# Autodesk Inventor assembly: V1Indexers
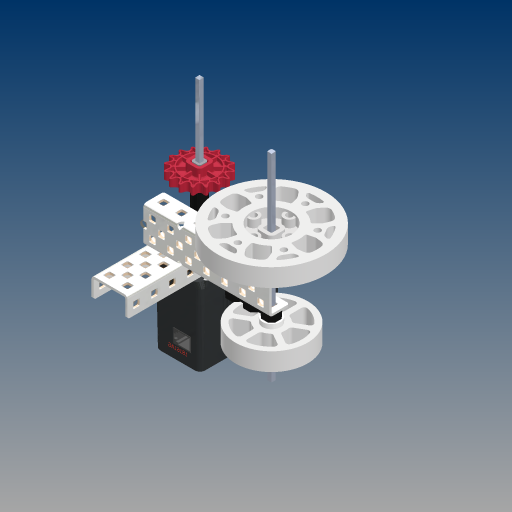
[picture p0: Inventor's stored thumbnail of the model, 512x512]
Saved by Autodesk Inventor 2023 (Build 270158000, 158)
## iProperties
Created: 2023-07-14
Part Number: V1Indexers
Document SubType Name: Assembly
Designer: eddie
Author: eddie
## Documents named in this file (20)
- C:\Users\eddie\Documents\81208X-Over-Under-CAD\V1\V1Indexer_Right.iam
- C:\Users\eddie\Documents\81208X-Over-Under-CAD\VEX-CAD-Inventor-1.4.0\Motion\Shaft LS\Shaft LS.ipt
- C:\Users\eddie\Documents\81208X-Over-Under-CAD\VEX-CAD-Inventor-1.4.0\Motion\Spacers\Spacer Nylon .375 OD\NSpacer .375 OD x .500.ipt
- C:\Users\eddie\Documents\81208X-Over-Under-CAD\VEX-CAD-Inventor-1.4.0\Motion\Spacers\Spacer Nylon .375 OD.ipt
- C:\Users\eddie\Documents\81208X-Over-Under-CAD\VEX-CAD-Inventor-1.4.0\Motion\Shaft LS\Shaft LS\Shaft LS 3.5.ipt
- C:\Users\eddie\Documents\81208X-Over-Under-CAD\VEX-CAD-Inventor-1.4.0\Motion\Shaft LS\Shaft LS\Shaft LS 5.5.ipt
- C:\Users\eddie\Documents\81208X-Over-Under-CAD\VEX-CAD-Inventor-1.4.0\Motion\Spacers\Spacer Nylon .500 OD\NSpacer White .500 OD x .125.ipt
- C:\Users\eddie\Documents\81208X-Over-Under-CAD\VEX-CAD-Inventor-1.4.0\Motion\Spacers\Spacer Nylon .500 OD.ipt
- C:\Users\eddie\Documents\81208X-Over-Under-CAD\VEX-CAD-Inventor-1.4.0\Motion\Wheels\Flex Wheels\2.000 Flex Wheel\2.000 30A .500.ipt
- C:\Users\eddie\Documents\81208X-Over-Under-CAD\VEX-CAD-Inventor-1.4.0\Motion\Wheels\Flex Wheels\2.000 Flex Wheel.ipt
- C:\Users\eddie\Documents\81208X-Over-Under-CAD\VEX-CAD-Inventor-1.4.0\Motion\Wheels\Flex Wheels\3.000 Flex Wheel\3.000 30A .500.ipt
- C:\Users\eddie\Documents\81208X-Over-Under-CAD\VEX-CAD-Inventor-1.4.0\Motion\Wheels\Flex Wheels\3.000 Flex Wheel.ipt
- C:\Users\eddie\Documents\81208X-Over-Under-CAD\VEX-CAD-Inventor-1.4.0\Structure\C Channel\Aluminum 1x2x1\Alu C 1x2x1x9_MIR1.ipt
- C:\Users\eddie\Documents\81208X-Over-Under-CAD\VEX-CAD-Inventor-1.4.0\Motion\Shaft LS\Bearing Flat_MIR2.ipt
- C:\Users\eddie\Documents\81208X-Over-Under-CAD\VEX-CAD-Inventor-1.4.0\Structure\C Channel\Aluminum 1x2x1\Alu C 1x2x1x7_MIR1.ipt
- C:\Users\eddie\Documents\81208X-Over-Under-CAD\VEX-CAD-Inventor-1.4.0\Electronics\V5 Motor_MIR1.ipt
- C:\Users\eddie\Documents\81208X-Over-Under-CAD\VEX-CAD-Inventor-1.4.0\Motion\Sprockets\6P Sprocket\6P 16T Sprocket, Square_MIR1.iam
- C:\Users\eddie\Documents\81208X-Over-Under-CAD\VEX-CAD-Inventor-1.4.0\Motion\Sprockets\6P Sprocket\6P 8T Sprocket, Square_MIR1.iam
- C:\Users\eddie\Documents\81208X-Over-Under-CAD\VEX-CAD-Inventor-1.4.0\Motion\Gears\HS Gear\HS 12T Gear, Square_MIR1.iam
- C:\Users\eddie\Documents\81208X-Over-Under-CAD\Custom-parts\36T HS Gear Insert_MIR_MIR.ipt
## Components (17 placed, 14 different names)
1. Alu C 1x2x1x9_MIR1:1 — Insert:40, Insert:41
2. Bearing Flat_MIR2:1 — Insert:40, Insert:42, Insert:45, Insert:46
3. Alu C 1x2x1x7_MIR1:1 — Insert:41, Insert:43, Insert:44, Insert:49, Insert:51
4. V5 Motor_MIR1:1 — Insert:42
5. Shaft LS 5.5:4
6. Bearing Flat_MIR2:2 — Insert:43, Insert:44, Insert:50
7. Shaft LS 3.5:5 — Insert:45
8. NSpacer .375 OD x .500:5 — Insert:46, Insert:47
9. NSpacer .375 OD x .500:6 — Insert:47, Insert:48
10. 6P 16T Sprocket, Square_MIR1:1 [sub-assembly] — Insert:48
11. 6P 8T Sprocket, Square_MIR1:1 [sub-assembly] — Insert:49, Insert:54
12. NSpacer White .500 OD x .125:2 — Insert:50, Insert:52, Insert:53
13. Bearing Flat_MIR2:3 — Insert:51
14. 2.000 30A .500:2 — Insert:52
15. HS 12T Gear, Square_MIR1:1 [sub-assembly] — Insert:53
16. 3.000 30A .500:3 — Insert:54
17. 36T HS Gear Insert_MIR_MIR:1
## Relationships (15: Insert 15)
- Insert:40: Alu C 1x2x1x9_MIR1:1 ↔ Bearing Flat_MIR2:1
- Insert:41: Alu C 1x2x1x9_MIR1:1 ↔ Alu C 1x2x1x7_MIR1:1
- Insert:42: Bearing Flat_MIR2:1 ↔ V5 Motor_MIR1:1
- Insert:43: Alu C 1x2x1x7_MIR1:1 ↔ Bearing Flat_MIR2:2
- Insert:44: Alu C 1x2x1x7_MIR1:1 ↔ Bearing Flat_MIR2:2
- Insert:45: Bearing Flat_MIR2:1 ↔ Shaft LS 3.5:5
- Insert:46: Bearing Flat_MIR2:1 ↔ NSpacer .375 OD x .500:5
- Insert:47: NSpacer .375 OD x .500:5 ↔ NSpacer .375 OD x .500:6
- Insert:48: NSpacer .375 OD x .500:6 ↔ 6P 16T Sprocket, Square_MIR1:1
- Insert:49: Alu C 1x2x1x7_MIR1:1 ↔ 6P 8T Sprocket, Square_MIR1:1
- Insert:50: Bearing Flat_MIR2:2 ↔ NSpacer White .500 OD x .125:2
- Insert:51: Alu C 1x2x1x7_MIR1:1 ↔ Bearing Flat_MIR2:3
- Insert:52: NSpacer White .500 OD x .125:2 ↔ 2.000 30A .500:2
- Insert:53: NSpacer White .500 OD x .125:2 ↔ HS 12T Gear, Square_MIR1:1
- Insert:54: 6P 8T Sprocket, Square_MIR1:1 ↔ 3.000 30A .500:3
